# Autodesk Inventor assembly: CoverPlate
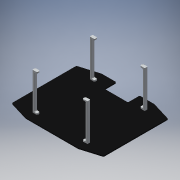
[picture p0: Inventor's stored thumbnail of the model, 180x180]
Saved by Autodesk Inventor 2016 (Build 200138000, 138)
## iProperties
Created: 2016-11-01
Part Number: CoverPlate
Document SubType Name: Assembly
Designer: lachesis
Author: lachesis
## Documents named in this file (4)
- C:\Users\lachesis\git\Swarmathon-Robot\CAD-Files\Assemblies\CoverPlate.iam
- C:\Users\lachesis\git\Swarmathon-Robot\CAD-Files\Parts\CoverPlate.ipt
- C:\Users\lachesis\git\Swarmathon-Robot\CAD-Files\Parts\LidSupport.ipt
- C:\Users\lachesis\git\Swarmathon-Robot\CAD-Files\Assemblies\CoverPlate_Substitute_1.ipt
## Components (6 placed, 3 different names)
1. CoverPlate:1 — Mate:1, Mate:2, Mate:3, Mate:4, Mate:5, Mate:6, Mate:7, Mate:8
2. LidSupport:1 — Mate:4, Mate:6
3. LidSupport:2 — Mate:3, Mate:8
4. LidSupport:3 — Mate:2, Mate:7
5. LidSupport:4 — Mate:1, Mate:5
6. CoverPlate_Substitute_1:1
## Relationships (8: Mate 8)
- Mate:1: CoverPlate:1 ↔ LidSupport:4
- Mate:2: CoverPlate:1 ↔ LidSupport:3
- Mate:3: CoverPlate:1 ↔ LidSupport:2
- Mate:4: CoverPlate:1 ↔ LidSupport:1
- Mate:5: CoverPlate:1 ↔ LidSupport:4
- Mate:6: CoverPlate:1 ↔ LidSupport:1
- Mate:7: CoverPlate:1 ↔ LidSupport:3
- Mate:8: CoverPlate:1 ↔ LidSupport:2
